# Autodesk Inventor assembly: Tamale Assembly Plate Assembly V3
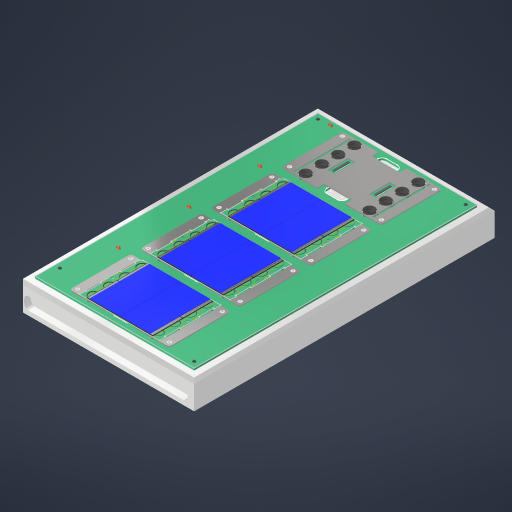
[picture p0: Inventor's stored thumbnail of the model, 512x512]
Saved by Autodesk Inventor 2024 (Build 280153000, 153)
## iProperties
Created: 2022-03-23
Part Number: Tamale Assembly Plate Assembly V3
Document SubType Name: Assembly
Designer: Caleb
Author: Caleb
## Documents named in this file (8)
- C:\Users\cfangmeier3\Desktop\nebraska-silicon-lab\Hardware\ETL\Module Assembly\Tamale Assembly Plate V5\Tamale Assembly Plate Assembly V5.iam
- C:\Users\cfangmeier3\Desktop\nebraska-silicon-lab\Hardware\ETL\Module Assembly\Tamale Assembly Plate V5\Tamale Assembly Plate V5.ipt
- C:\Users\cfangmeier3\Desktop\nebraska-silicon-lab\Hardware\ETL\Module Assembly\Tamale Assembly Plate V5\spacer V5.ipt
- C:\Users\cfangmeier3\Desktop\nebraska-silicon-lab\Hardware\ETL\Module Assembly\Tamale Assembly Plate V5\91771A054_Passivated 18-8 Stainless Steel Phillips Flat Head Screw.ipt
- C:\Users\cfangmeier3\Desktop\nebraska-silicon-lab\Hardware\ETL\Module Assembly\Tamale Assembly Plate V5\90910A443_BUTTON HEAD TORX SCREWS.ipt
- C:\Users\cfangmeier3\Desktop\nebraska-silicon-lab\Hardware\ETL\Module Assembly\Tamale Assembly Plate V5\5427A604_Vacuum Cup.ipt
- C:\Users\cfangmeier3\Desktop\nebraska-silicon-lab\Hardware\ETL\Module Assembly\Tamale Assembly Plate V5\etl_assembly_plate_pcb_v5.ipt
- C:\Users\cfangmeier3\Desktop\nebraska-silicon-lab\Hardware\ETL\modules\tamale v1.5\Tamale - V1p5.iam
## Components (62 placed, 7 different names)
1. Tamale Assembly Plate V5:1 — Insert:16, Insert:17, Angle:2, Angle:3, Insert:18, Insert:19, Insert:20, Insert:21, Insert:22, Insert:23
2. 90910A443_BUTTON HEAD TORX SCREWS:1
3. 90910A443_BUTTON HEAD TORX SCREWS:2
4. 90910A443_BUTTON HEAD TORX SCREWS:3
5. 90910A443_BUTTON HEAD TORX SCREWS:4
6. etl_assembly_plate_pcb_v5:1 — Insert:24
7. 91771A054_Passivated 18-8 Stainless Steel Phillips Flat Head Screw:4 — Insert:28
8. spacer V5:1 — Mate:3, Flush:1, Insert:24, Insert:25, Insert:26, Insert:27, Insert:28, Flush:2
9. 91771A054_Passivated 18-8 Stainless Steel Phillips Flat Head Screw:3 — Insert:27
10. Tamale - V1p5:1 [sub-assembly] — Angle:2, Angle:3, Mate:3, Flush:1, Flush:2
11. 91771A054_Passivated 18-8 Stainless Steel Phillips Flat Head Screw:2 — Insert:26
12. 91771A054_Passivated 18-8 Stainless Steel Phillips Flat Head Screw:1 — Insert:25
13. 5427A604_Vacuum Cup:8 — Insert:20
14. 5427A604_Vacuum Cup:7 — Insert:21
15. 5427A604_Vacuum Cup:6 — Insert:22
16. 5427A604_Vacuum Cup:5 — Insert:23
17. 5427A604_Vacuum Cup:4 — Insert:19
18. 5427A604_Vacuum Cup:3 — Insert:18
19. 5427A604_Vacuum Cup:2 — Insert:17
20. 5427A604_Vacuum Cup:1 — Insert:16
21. 91771A054_Passivated 18-8 Stainless Steel Phillips Flat Head Screw:5
22. spacer V5:2
23. 91771A054_Passivated 18-8 Stainless Steel Phillips Flat Head Screw:6
24. Tamale - V1p5:2 [sub-assembly]
25. 91771A054_Passivated 18-8 Stainless Steel Phillips Flat Head Screw:7
26. 91771A054_Passivated 18-8 Stainless Steel Phillips Flat Head Screw:8
27. 5427A604_Vacuum Cup:9
28. 5427A604_Vacuum Cup:10
29. 5427A604_Vacuum Cup:11
30. 5427A604_Vacuum Cup:12
31. 5427A604_Vacuum Cup:13
32. 5427A604_Vacuum Cup:14
33. 5427A604_Vacuum Cup:15
34. 5427A604_Vacuum Cup:16
35. 91771A054_Passivated 18-8 Stainless Steel Phillips Flat Head Screw:9
36. spacer V5:3
37. 91771A054_Passivated 18-8 Stainless Steel Phillips Flat Head Screw:10
38. Tamale - V1p5:3 [sub-assembly]
39. 91771A054_Passivated 18-8 Stainless Steel Phillips Flat Head Screw:11
40. 91771A054_Passivated 18-8 Stainless Steel Phillips Flat Head Screw:12
41. 5427A604_Vacuum Cup:17
42. 5427A604_Vacuum Cup:18
43. 5427A604_Vacuum Cup:19
44. 5427A604_Vacuum Cup:20
45. 5427A604_Vacuum Cup:21
46. 5427A604_Vacuum Cup:22
47. 5427A604_Vacuum Cup:23
48. 5427A604_Vacuum Cup:24
49. 91771A054_Passivated 18-8 Stainless Steel Phillips Flat Head Screw:13
50. spacer V5:4
51. 91771A054_Passivated 18-8 Stainless Steel Phillips Flat Head Screw:14
52. Tamale - V1p5:4 [sub-assembly]
53. 91771A054_Passivated 18-8 Stainless Steel Phillips Flat Head Screw:15
54. 91771A054_Passivated 18-8 Stainless Steel Phillips Flat Head Screw:16
55. 5427A604_Vacuum Cup:25
56. 5427A604_Vacuum Cup:26
57. 5427A604_Vacuum Cup:27
58. 5427A604_Vacuum Cup:28
59. 5427A604_Vacuum Cup:29
60. 5427A604_Vacuum Cup:30
61. 5427A604_Vacuum Cup:31
62. 5427A604_Vacuum Cup:32
## Component patterns: (4 elements, first: 91771A054_Passivated 18-8 Stainless Steel Phillips Flat Head Screw:4 + spacer V5:1 + 91771A054_Passivated 18-8 Stainless Steel Phillips Flat Head Screw:3 + Tamale - V1p5:1 + 91771A054_Passivated 18-8 Stainless Steel Phillips Flat Head Screw:2 + 91771A054_Passivated 18-8 Stainless Steel Phillips Flat Head Screw:1 + 5427A604_Vacuum Cup:8 + 5427A604_Vacuum Cup:7 + 5427A604_Vacuum Cup:6 + 5427A604_Vacuum Cup:5 + 5427A604_Vacuum Cup:4 + 5427A604_Vacuum Cup:3 + 5427A604_Vacuum Cup:2 + 5427A604_Vacuum Cup:1)
## Relationships (21: Insert 14, Angle 3, Mate 2, Flush 2)
- [Insert]: Tamale Assembly Plate V5:1 ↔ etl_assembly_plate_pcb_v5:1
- Insert:16: Tamale Assembly Plate V5:1 ↔ 5427A604_Vacuum Cup:1
- [Angle] (0 deg): Tamale Assembly Plate V5:1 ↔ etl_assembly_plate_pcb_v5:1
- [Mate]: etl_assembly_plate_pcb_v5:1 ↔ spacer V5:1
- Insert:17: Tamale Assembly Plate V5:1 ↔ 5427A604_Vacuum Cup:2
- Angle:2 (0 deg): Tamale Assembly Plate V5:1 ↔ Tamale - V1p5:1
- Angle:3 (0 deg): Tamale Assembly Plate V5:1 ↔ Tamale - V1p5:1
- Insert:18: Tamale Assembly Plate V5:1 ↔ 5427A604_Vacuum Cup:3
- Insert:19: Tamale Assembly Plate V5:1 ↔ 5427A604_Vacuum Cup:4
- Insert:20: Tamale Assembly Plate V5:1 ↔ 5427A604_Vacuum Cup:8
- Insert:21: Tamale Assembly Plate V5:1 ↔ 5427A604_Vacuum Cup:7
- Insert:22: Tamale Assembly Plate V5:1 ↔ 5427A604_Vacuum Cup:6
- Insert:23: Tamale Assembly Plate V5:1 ↔ 5427A604_Vacuum Cup:5
- Mate:3: spacer V5:1 ↔ Tamale - V1p5:1
- Flush:1: spacer V5:1 ↔ Tamale - V1p5:1
- Insert:24: etl_assembly_plate_pcb_v5:1 ↔ spacer V5:1
- Insert:25: spacer V5:1 ↔ 91771A054_Passivated 18-8 Stainless Steel Phillips Flat Head Screw:1
- Insert:26: spacer V5:1 ↔ 91771A054_Passivated 18-8 Stainless Steel Phillips Flat Head Screw:2
- Insert:27: spacer V5:1 ↔ 91771A054_Passivated 18-8 Stainless Steel Phillips Flat Head Screw:3
- Insert:28: 91771A054_Passivated 18-8 Stainless Steel Phillips Flat Head Screw:4 ↔ spacer V5:1
- Flush:2 (7 mm): spacer V5:1 ↔ Tamale - V1p5:1
